# Autodesk Inventor assembly: z_axys
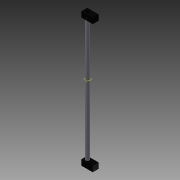
[picture p0: Inventor's stored thumbnail of the model, 180x180]
Saved by Autodesk Inventor 2014 SP1 (Build 180222100, 222)
## iProperties
Created: 2015-04-08
Part Number: z_axys
Document SubType Name: Assembly
Designer: Giorgio Nuzzo
Author: Giorgio Nuzzo
## Documents named in this file (5)
- C:\Users\Giorgio Nuzzo\Desktop\3dragmodel\z_axys.iam
- C:\Users\Giorgio Nuzzo\Desktop\3dragmodel\supporto_guide_10Z.ipt
- C:\Users\Giorgio Nuzzo\Desktop\3dragmodel\guida_Z.ipt
- C:\Users\Giorgio Nuzzo\Desktop\3dragmodel\supporto_guide_10Z_MIR.ipt
- C:\Users\Giorgio Nuzzo\Desktop\3dragmodel\guida__Z.ipt
## Components (4 placed, 4 different names)
1. supporto_guide_10Z:1 — Mate:1, Flush:1
2. guida_Z:1 — Flush:1, Flush:2
3. supporto_guide_10Z_MIR:1 — Mate:2
4. guida__Z:1 — Flush:2
## Relationships (4: Mate 2, Flush 2)
- Mate:1: supporto_guide_10Z:1
- Flush:1: supporto_guide_10Z:1 ↔ guida_Z:1
- Mate:2: supporto_guide_10Z_MIR:1
- Flush:2: guida_Z:1 ↔ guida__Z:1
